# Autodesk Inventor assembly: Arm_Shim
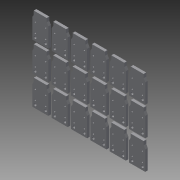
[picture p0: Inventor's stored thumbnail of the model, 180x180]
Saved by Autodesk Inventor 2013 (Build 170138000, 138)
## iProperties
Created: 2014-05-16
Part Number: Arm_Shim
Document SubType Name: Assembly
Designer: andou
Author: andou
## Documents named in this file (2)
- C:\Users\andou\Documents\Inventor\RoboticsProject\project_4\Robot\CNC\Arm_Link_Shim_18.iam
- C:\Users\andou\Documents\Inventor\RoboticsProject\project_4\Robot\CNC\Arm_Link_Shim_i.ipt
## Components (18 placed, 1 different names)
1. Arm_Link_Shim_i:1
2. Arm_Link_Shim_i:2
3. Arm_Link_Shim_i:3
4. Arm_Link_Shim_i:4
5. Arm_Link_Shim_i:5
6. Arm_Link_Shim_i:6
7. Arm_Link_Shim_i:7
8. Arm_Link_Shim_i:8
9. Arm_Link_Shim_i:9
10. Arm_Link_Shim_i:10
11. Arm_Link_Shim_i:11
12. Arm_Link_Shim_i:12
13. Arm_Link_Shim_i:13
14. Arm_Link_Shim_i:14
15. Arm_Link_Shim_i:15
16. Arm_Link_Shim_i:16
17. Arm_Link_Shim_i:17
18. Arm_Link_Shim_i:18
## Component patterns: (18 elements, first: Arm_Link_Shim_i:1)
